# Autodesk Inventor assembly: 4x2020_in
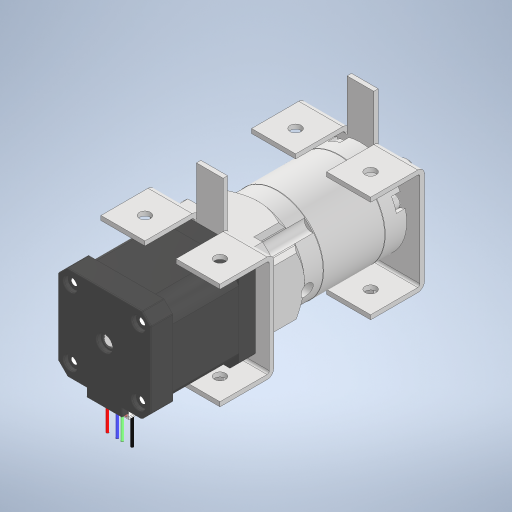
[picture p0: Inventor's stored thumbnail of the model, 512x512]
Saved by Autodesk Inventor 2024 (Build 280153000, 153)
## iProperties
Created: 2025-12-16
Part Number: 4x2020_in
Document SubType Name: Assembly
Designer: schar
Author: schar
## Documents named in this file (5)
- C:\Users\schar\Desktop\projectBlueprint\AMSTS\hardware\4x2020_in.iam
- C:\Users\schar\Desktop\projectBlueprint\AMSTS\hardware\4x2020_universal.ipt
- C:\Users\schar\Desktop\projectBlueprint\AMSTS\hardware\17HE19-2004S.ipt
- C:\Users\schar\Desktop\projectBlueprint\AMSTS\hardware\4x2020_universal_planetary.ipt
- C:\Users\schar\Desktop\projectBlueprint\AMSTS\hardware\EG17-G20.iam
## Components (4 placed, 4 different names)
1. 4x2020_universal:1 — Mate:1, Mate:2, Mate:3, Mate:4, Mate:5, Mate:6
2. 17HE19-2004S:1 — Mate:1, Mate:2, Mate:3
3. 4x2020_universal_planetary:1 — Mate:7, Mate:8, Mate:9
4. EG17-G20:1 [sub-assembly] — Mate:4, Mate:5, Mate:6, Mate:7, Mate:8, Mate:9
## Relationships (9: Mate 9)
- Mate:1: 4x2020_universal:1 ↔ 17HE19-2004S:1
- Mate:2: 4x2020_universal:1 ↔ 17HE19-2004S:1
- Mate:3: 4x2020_universal:1 ↔ 17HE19-2004S:1
- Mate:4: 4x2020_universal:1 ↔ EG17-G20:1
- Mate:5: 4x2020_universal:1 ↔ EG17-G20:1
- Mate:6: 4x2020_universal:1 ↔ EG17-G20:1
- Mate:7: 4x2020_universal_planetary:1 ↔ EG17-G20:1
- Mate:8: 4x2020_universal_planetary:1 ↔ EG17-G20:1
- Mate:9: 4x2020_universal_planetary:1 ↔ EG17-G20:1
